# Autodesk Inventor assembly: bit bot top assembly
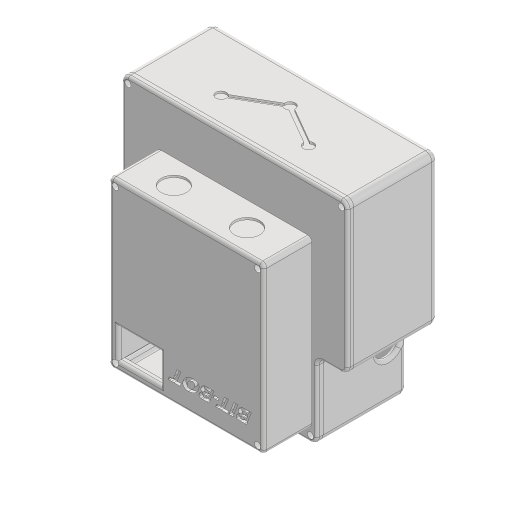
[picture p0: Inventor's stored thumbnail of the model, 512x512]
Saved by Autodesk Inventor 2024 (Build 280153000, 153)
## iProperties
Created: 2024-01-27
Part Number: bit bot top assembly
Document SubType Name: Assembly
Designer: chris
Author: chris
## Documents named in this file (4)
- C:\Users\chris\Desktop\STL files\bit-bot\bit bot top assembly.iam
- C:\Users\chris\Desktop\STL files\bit-bot\bit_bot_top.ipt
- C:\Users\chris\Desktop\STL files\bit-bot\bit bot lid 1.ipt
- C:\Users\chris\Desktop\STL files\bit-bot\bit bot battery pack.ipt
## Components (3 placed, 3 different names)
1. bit_bot_top:1 — Rotational:1, Flush:1
2. bit bot lid 1:1 — Rotational:1, Flush:1, Rotational:2, Rotational:3
3. bit bot battery pack:1 — Rotational:2, Rotational:3
## Relationships (4: RevoluteJoint 3, Flush 1)
- Rotational:1 [RevoluteJoint]: bit_bot_top:1 ↔ bit bot lid 1:1
- Flush:1: bit_bot_top:1 ↔ bit bot lid 1:1
- Rotational:2 [RevoluteJoint]: bit bot lid 1:1 ↔ bit bot battery pack:1
- Rotational:3 [RevoluteJoint]: bit bot lid 1:1 ↔ bit bot battery pack:1
